# Autodesk Inventor assembly: 15102898-16-A-0400
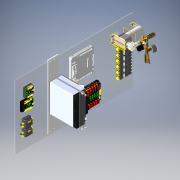
[picture p0: Inventor's stored thumbnail of the model, 180x180]
Saved by Autodesk Inventor 2017 (Build 210142000, 142)
## iProperties
Created: 2016-10-03
Part Number: 15102898-16-A-0400
Document SubType Name: Assembly
Designer: gus
Mass: 5100.32 g
Surface Area: 9058.32 cm^2
Volume: 4409.06 cm^3
Density: 1.15678 g/cm^3
Author: gus
## Documents named in this file (23)
- \\Mac\Home\Desktop\bunnybots 2016\15102898-16-Bunnybot-CAD\Bunnybot-To_be_renamed\15102898-16-A-0000\15102898-16-A-0400\15102898-16-A-0400.iam
- \\Mac\Home\Desktop\bunnybots 2016\15102898-16-Bunnybot-CAD\Bunnybot-To_be_renamed\15102898-16-A-0000\15102898-16-A-0400\15102898-16-P-0401.ipt
- \\Mac\Home\Desktop\bunnybots 2016\15102898-16-Bunnybot-CAD\Bunnybot-To_be_renamed\15102898-16-A-0000\15102898-16-A-0400\Imported Components\User Library-Battery-6.ipt
- \\Mac\Home\Desktop\bunnybots 2016\15102898-16-Bunnybot-CAD\Bunnybot-To_be_renamed\15102898-16-A-0000\15102898-16-A-0400\15102898-16-P-0402.ipt
- \\Mac\Home\Desktop\bunnybots 2016\15102898-16-Bunnybot-CAD\Bunnybot-To_be_renamed\15102898-16-A-0000\15102898-16-A-0400\15102898-16-P-0403.ipt
- \\Mac\Home\Desktop\bunnybots 2016\15102898-16-Bunnybot-CAD\Bunnybot-To_be_renamed\15102898-16-A-0000\15102898-16-A-0400\15102898-16-P-0404.ipt
- \\Mac\Home\Desktop\bunnybots 2016\15102898-16-Bunnybot-CAD\Bunnybot-To_be_renamed\15102898-16-A-0000\15102898-16-A-0400\15102898-16-P-0405.ipt
- \\Mac\Home\Desktop\bunnybots 2016\15102898-16-Bunnybot-CAD\Bunnybot-To_be_renamed\15102898-16-A-0000\15102898-16-A-0300\Imported Components\91860A029_TYPE 17-7 PH STAINLESS STEEL FLAT WASHER.ipt
- \\Mac\Home\Desktop\bunnybots 2016\15102898-16-Bunnybot-CAD\Bunnybot-To_be_renamed\15102898-16-A-0000\15102898-16-A-0300\Imported Components\92001A321_18-8 SS WING NUT.ipt
- \\Mac\Home\Desktop\bunnybots 2016\15102898-16-Bunnybot-CAD\Bunnybot-To_be_renamed\15102898-16-A-0000\15102898-16-A-0400\Imported Components\217-0220-STEP.ipt
- \\Mac\Home\Desktop\bunnybots 2016\15102898-16-Bunnybot-CAD\Bunnybot-To_be_renamed\15102898-16-A-0000\15102898-16-A-0400\Imported Components\Imported Components\217-4243\217-4243.ipt
- \\Mac\Home\Desktop\bunnybots 2016\15102898-16-Bunnybot-CAD\Bunnybot-To_be_renamed\15102898-16-A-0000\15102898-16-A-0400\Imported Components\Imported Components\217-4244\217-4244.ipt
- \\Mac\Home\Desktop\bunnybots 2016\15102898-16-Bunnybot-CAD\Bunnybot-To_be_renamed\15102898-16-A-0000\15102898-16-A-0400\Imported Components\Imported Components\217-4245\217-4245.ipt
- \\Mac\Home\Desktop\bunnybots 2016\15102898-16-Bunnybot-CAD\Bunnybot-To_be_renamed\15102898-16-A-0000\15102898-16-A-0400\Imported Components\Imported Components\217-8080-STEP-20150925 No wires\217-8080-STEP-20150925.iam
- \\Mac\Home\Desktop\bunnybots 2016\15102898-16-Bunnybot-CAD\Bunnybot-To_be_renamed\15102898-16-A-0000\15102898-16-A-0400\Imported Components\Imported Components\cd_roborio\cd_roborio.ipt
- \\Mac\Home\Desktop\bunnybots 2016\15102898-16-Bunnybot-CAD\Bunnybot-To_be_renamed\15102898-16-A-0000\15102898-16-A-0400\Imported Components\Pneu_Compressor_0090C.iam
- \\Mac\Home\Desktop\bunnybots 2016\15102898-16-Bunnybot-CAD\Bunnybot-To_be_renamed\15102898-16-A-0000\15102898-16-A-0400\Imported Components\Pneu_Norgren_16-004-011.ipt
- \\Mac\Home\Desktop\bunnybots 2016\15102898-16-Bunnybot-CAD\Bunnybot-To_be_renamed\15102898-16-A-0000\15102898-16-A-0400\Imported Components\Pneu_UnionTee_2203P-2.ipt
- \\Mac\Home\Desktop\bunnybots 2016\15102898-16-Bunnybot-CAD\Bunnybot-To_be_renamed\15102898-16-A-0000\15102898-16-A-0400\Imported Components\Pneu_Connector_w68plp-4-2.ipt
- \\Mac\Home\Desktop\bunnybots 2016\15102898-16-Bunnybot-CAD\Bunnybot-To_be_renamed\15102898-16-A-0000\15102898-16-A-0400\Imported Components\Pneu_Nipple_216P-2.ipt
- \\Mac\Home\Desktop\bunnybots 2016\15102898-16-Bunnybot-CAD\Bunnybot-To_be_renamed\15102898-16-A-0000\15102898-16-A-0400\Imported Components\Pneu_Switch_SM-2B-115R.ipt
- \\Mac\Home\Desktop\bunnybots 2016\15102898-16-Bunnybot-CAD\Bunnybot-To_be_renamed\15102898-16-A-0000\15102898-16-A-0400\Imported Components\Pneu_Norgren_18-013-212.iam
- \\Mac\Home\Desktop\bunnybots 2016\15102898-16-Bunnybot-CAD\Bunnybot-To_be_renamed\15102898-16-A-0000\15102898-16-A-0400\Imported Components\parts\Pneu_Parker_MV709-2.ipt
## Components (37 placed, 22 different names)
1. 15102898-16-P-0401:1 — Flush:1, Flush:2, Mate:1, Mate:4, Flush:4, Flush:5, Mate:18, Mate:19, Mate:20, Mate:21, Mate:22, Mate:23, Mate:24
2. User Library-Battery-6:1 — Flush:1, Flush:2, Mate:2, Flush:3, Mate:3, Mate:7
3. 15102898-16-P-0402:1 — Mate:1, Mate:2, Flush:3, Mate:3, Angle:1
4. 15102898-16-P-0403:1 — Mate:4, Flush:4, Flush:5, Mate:5, Flush:6, Mate:6, Flush:7
5. 15102898-16-P-0404:1 — Mate:5, Flush:6, Mate:9, Mate:13, Mate:15
6. 15102898-16-P-0404:2 — Mate:6, Flush:7, Mate:8, Mate:11, Mate:17
7. 15102898-16-P-0405:1 — Mate:7, Mate:8, Mate:9, Mate:10, Mate:12, Mate:14, Mate:16
8. 91860A029_TYPE 17-7 PH STAINLESS STEEL FLAT WASHER:1 — Mate:12, Mate:13
9. 92001A321_18-8 SS WING NUT:1 — Mate:16, Mate:17
10. 91860A029_TYPE 17-7 PH STAINLESS STEEL FLAT WASHER:2 — Mate:10, Mate:11
11. 92001A321_18-8 SS WING NUT:2 — Mate:14, Mate:15
12. 217-4243:1 — Mate:22
13. 217-4244:1 — Mate:18, Angle:1
14. 217-4245:1 — Mate:21
15. cd_roborio:1 — Mate:19
16. Pneu_Compressor_0090C:1 [sub-assembly] — Mate:24, Mate:25, Mate:26
17. Pneu_Norgren_16-004-011:1 — Insert:3
18. Pneu_UnionTee_2203P-2:1 — Mate:25, Mate:26, Mate:29, Mate:30, Insert:1, Flush:8
19. Pneu_Connector_w68plp-4-2:1 — Mate:29, Mate:30
20. Pneu_Nipple_216P-2:1 — Insert:1, Insert:2
21. Pneu_UnionTee_2203P-2:2 — Insert:2, Insert:3, Insert:4, Flush:8, Flush:10
22. Pneu_Nipple_216P-2:2 — Insert:4, Insert:5
23. Pneu_UnionTee_2203P-2:3 — Insert:5, Insert:6, Insert:7, Flush:10
24. Pneu_Switch_SM-2B-115R:1 — Insert:6
25. Pneu_Nipple_216P-2:3 — Insert:7, Insert:8
26. Pneu_UnionTee_2203P-2:4 — Insert:8, Insert:9, Insert:10
27. Pneu_Norgren_18-013-212:1 [sub-assembly] — Insert:9
28. Pneu_Nipple_216P-2:4 — Insert:10, Insert:11
29. Pneu_Parker_MV709-2:1 — Insert:11
30. 217-8080-STEP-20150925:1 [sub-assembly] — Mate:20
31. 217-8080-STEP-20150925:2 [sub-assembly]
32. 217-8080-STEP-20150925:3 [sub-assembly]
33. 217-8080-STEP-20150925:4 [sub-assembly]
34. 217-8080-STEP-20150925:5 [sub-assembly]
35. 217-8080-STEP-20150925:6 [sub-assembly]
36. 217-0220-STEP:1 — Mate:23
37. 217-0220-STEP:2
## Component patterns: (6 elements, first: 217-8080-STEP-20150925:1), (2 elements, first: 217-0220-STEP:1)
## Relationships (49: Mate 28, Insert 11, Flush 9, Angle 1)
- Flush:1 (215.9 mm): 15102898-16-P-0401:1 ↔ User Library-Battery-6:1
- Flush:2 (114.3 mm): 15102898-16-P-0401:1 ↔ User Library-Battery-6:1
- Mate:1: 15102898-16-P-0401:1 ↔ 15102898-16-P-0402:1
- Mate:2: User Library-Battery-6:1 ↔ 15102898-16-P-0402:1
- Flush:3: User Library-Battery-6:1 ↔ 15102898-16-P-0402:1
- Mate:3: User Library-Battery-6:1 ↔ 15102898-16-P-0402:1
- Mate:4: 15102898-16-P-0401:1 ↔ 15102898-16-P-0403:1
- Flush:4: 15102898-16-P-0401:1 ↔ 15102898-16-P-0403:1
- Flush:5 (214.3125 mm): 15102898-16-P-0401:1 ↔ 15102898-16-P-0403:1
- Mate:5: 15102898-16-P-0403:1 ↔ 15102898-16-P-0404:1
- Flush:6 (-6.35 mm): 15102898-16-P-0403:1 ↔ 15102898-16-P-0404:1
- Mate:6: 15102898-16-P-0403:1 ↔ 15102898-16-P-0404:2
- Flush:7 (-6.35 mm): 15102898-16-P-0403:1 ↔ 15102898-16-P-0404:2
- Mate:7: User Library-Battery-6:1 ↔ 15102898-16-P-0405:1
- Mate:8: 15102898-16-P-0404:2 ↔ 15102898-16-P-0405:1
- Mate:9: 15102898-16-P-0404:1 ↔ 15102898-16-P-0405:1
- Mate:10: 15102898-16-P-0405:1 ↔ 91860A029_TYPE 17-7 PH STAINLESS STEEL FLAT WASHER:2
- Mate:11: 15102898-16-P-0404:2 ↔ 91860A029_TYPE 17-7 PH STAINLESS STEEL FLAT WASHER:2
- Mate:12: 15102898-16-P-0405:1 ↔ 91860A029_TYPE 17-7 PH STAINLESS STEEL FLAT WASHER:1
- Mate:13: 15102898-16-P-0404:1 ↔ 91860A029_TYPE 17-7 PH STAINLESS STEEL FLAT WASHER:1
- Mate:14: 15102898-16-P-0405:1 ↔ 92001A321_18-8 SS WING NUT:2
- Mate:15: 15102898-16-P-0404:1 ↔ 92001A321_18-8 SS WING NUT:2
- Mate:16: 15102898-16-P-0405:1 ↔ 92001A321_18-8 SS WING NUT:1
- Mate:17: 15102898-16-P-0404:2 ↔ 92001A321_18-8 SS WING NUT:1
- Mate:18: 15102898-16-P-0401:1 ↔ 217-4244:1
- Angle:1 (90 deg): 15102898-16-P-0402:1 ↔ 217-4244:1
- Mate:19: 15102898-16-P-0401:1 ↔ cd_roborio:1
- Mate:20: 15102898-16-P-0401:1 ↔ 217-8080-STEP-20150925:1
- Mate:21: 15102898-16-P-0401:1 ↔ 217-4245:1
- Mate:22: 15102898-16-P-0401:1 ↔ 217-4243:1
- Mate:23: 15102898-16-P-0401:1 ↔ 217-0220-STEP:1
- Mate:24: 15102898-16-P-0401:1 ↔ Pneu_Compressor_0090C:1
- Mate:25: Pneu_Compressor_0090C:1 ↔ Pneu_UnionTee_2203P-2:1
- Mate:26: Pneu_Compressor_0090C:1 ↔ Pneu_UnionTee_2203P-2:1
- Mate:29: Pneu_UnionTee_2203P-2:1 ↔ Pneu_Connector_w68plp-4-2:1
- Mate:30: Pneu_UnionTee_2203P-2:1 ↔ Pneu_Connector_w68plp-4-2:1
- Insert:1: Pneu_UnionTee_2203P-2:1 ↔ Pneu_Nipple_216P-2:1
- Insert:2: Pneu_Nipple_216P-2:1 ↔ Pneu_UnionTee_2203P-2:2
- Insert:3: Pneu_Norgren_16-004-011:1 ↔ Pneu_UnionTee_2203P-2:2
- Insert:4: Pneu_UnionTee_2203P-2:2 ↔ Pneu_Nipple_216P-2:2
- Insert:5: Pneu_Nipple_216P-2:2 ↔ Pneu_UnionTee_2203P-2:3
- Insert:6: Pneu_UnionTee_2203P-2:3 ↔ Pneu_Switch_SM-2B-115R:1
- Flush:8: Pneu_UnionTee_2203P-2:1 ↔ Pneu_UnionTee_2203P-2:2
- Insert:7: Pneu_UnionTee_2203P-2:3 ↔ Pneu_Nipple_216P-2:3
- Insert:8: Pneu_Nipple_216P-2:3 ↔ Pneu_UnionTee_2203P-2:4
- Insert:9: Pneu_UnionTee_2203P-2:4 ↔ Pneu_Norgren_18-013-212:1
- Flush:10: Pneu_UnionTee_2203P-2:2 ↔ Pneu_UnionTee_2203P-2:3
- Insert:10: Pneu_UnionTee_2203P-2:4 ↔ Pneu_Nipple_216P-2:4
- Insert:11: Pneu_Nipple_216P-2:4 ↔ Pneu_Parker_MV709-2:1
